# Autodesk Inventor assembly: GP3-100
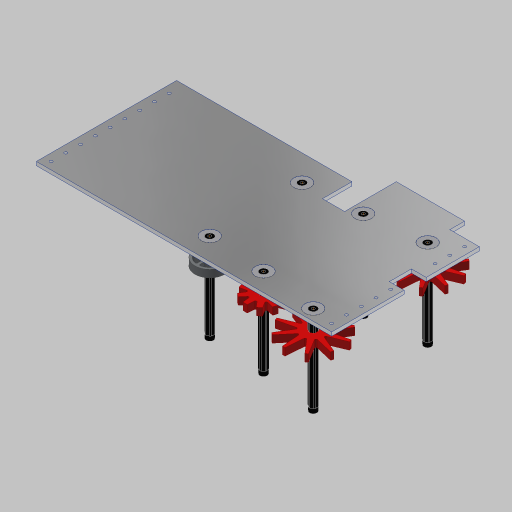
[picture p0: Inventor's stored thumbnail of the model, 512x512]
Saved by Autodesk Inventor 2023.5 (Build 275446000, 446)
## iProperties
Created: 2025-02-22
Part Number: GP3-100
Document SubType Name: Assembly
Designer: slick
Author: slick
## Documents named in this file (7)
- C:\Users\slick\OneDrive\Desktop\2025-ReefScape---CAD\ground intake\GP3\GP3-100.iam
- C:\Users\slick\OneDrive\Desktop\2025-ReefScape---CAD\ground intake\GP3\GP3-001.ipt
- C:\Users\slick\OneDrive\Desktop\2025-ReefScape---CAD\COMMON PARTS\BEARINGS\0_500_ID_x_1_125_OD_x_0_313_WD_Flanged_Bearing_217-2731.ipt
- C:\Users\slick\OneDrive\Desktop\2025-ReefScape---CAD\ground intake\GP3\GP3-002.ipt
- C:\Users\slick\OneDrive\Desktop\2025-ReefScape---CAD\COMMON PARTS\WHEELS\am-0619a .425 Hex Entrapption Star Cut to 4In.ipt
- C:\Users\slick\OneDrive\Desktop\2025-ReefScape---CAD\COMMON PARTS\WHEELS\am-0619a .425 Hex Entrapption Star Cut to 2 half In.ipt
- C:\Users\slick\OneDrive\Desktop\2025-ReefScape---CAD\COMMON PARTS\WHEELS\2_OD_Straight_Flex_Wheel_217-6354.ipt
## Components (19 placed, 6 different names)
1. GP3-001:1 — Insert:1, Insert:2, Insert:3, Mate:6, Insert:4, Insert:5, Insert:6
2. 0_500_ID_x_1_125_OD_x_0_313_WD_Flanged_Bearing_217-2731:1 — Insert:2, Mate:2, Flush:2
3. 0_500_ID_x_1_125_OD_x_0_313_WD_Flanged_Bearing_217-2731:2 — Insert:1, Mate:3, Flush:1
4. 0_500_ID_x_1_125_OD_x_0_313_WD_Flanged_Bearing_217-2731:3 — Insert:3, Mate:1, Flush:3
5. GP3-002:1 — Mate:3, Flush:1, Mate:5
6. GP3-002:2 — Mate:1, Flush:3, Mate:4
7. GP3-002:3 — Mate:2, Flush:2, Mate:8
8. am-0619a .425 Hex Entrapption Star Cut to 4In:2 — Mate:5, Flush:4
9. am-0619a .425 Hex Entrapption Star Cut to 4In:1 — Mate:4, Flush:4, Mate:6, Flush:7
10. 0_500_ID_x_1_125_OD_x_0_313_WD_Flanged_Bearing_217-2731:4 — Insert:4
11. GP3-002:4 — Mate:9
12. am-0619a .425 Hex Entrapption Star Cut to 2 half In:1 — Mate:8, Flush:6
13. am-0619a .425 Hex Entrapption Star Cut to 2 half In:2 — Mate:9, Flush:6, Flush:7, Flush:11
14. 0_500_ID_x_1_125_OD_x_0_313_WD_Flanged_Bearing_217-2731:5 — Insert:5
15. GP3-002:5 — Mate:12
16. 0_500_ID_x_1_125_OD_x_0_313_WD_Flanged_Bearing_217-2731:6 — Insert:6
17. GP3-002:6 — Mate:13
18. 2_OD_Straight_Flex_Wheel_217-6354:1 — Mate:13, Flush:10
19. 2_OD_Straight_Flex_Wheel_217-6354:2 — Mate:12, Flush:10, Flush:11
## Relationships (30: Mate 13, Flush 11, Insert 6)
- Insert:1: GP3-001:1 ↔ 0_500_ID_x_1_125_OD_x_0_313_WD_Flanged_Bearing_217-2731:2
- Insert:2: GP3-001:1 ↔ 0_500_ID_x_1_125_OD_x_0_313_WD_Flanged_Bearing_217-2731:1
- Insert:3: GP3-001:1 ↔ 0_500_ID_x_1_125_OD_x_0_313_WD_Flanged_Bearing_217-2731:3
- Mate:1: 0_500_ID_x_1_125_OD_x_0_313_WD_Flanged_Bearing_217-2731:3 ↔ GP3-002:2
- Mate:2: 0_500_ID_x_1_125_OD_x_0_313_WD_Flanged_Bearing_217-2731:1 ↔ GP3-002:3
- Mate:3: 0_500_ID_x_1_125_OD_x_0_313_WD_Flanged_Bearing_217-2731:2 ↔ GP3-002:1
- Flush:1: 0_500_ID_x_1_125_OD_x_0_313_WD_Flanged_Bearing_217-2731:2 ↔ GP3-002:1
- Flush:2: 0_500_ID_x_1_125_OD_x_0_313_WD_Flanged_Bearing_217-2731:1 ↔ GP3-002:3
- Flush:3: 0_500_ID_x_1_125_OD_x_0_313_WD_Flanged_Bearing_217-2731:3 ↔ GP3-002:2
- Mate:4: GP3-002:2 ↔ am-0619a .425 Hex Entrapption Star Cut to 4In:1
- Mate:5: GP3-002:1 ↔ am-0619a .425 Hex Entrapption Star Cut to 4In:2
- Flush:4: am-0619a .425 Hex Entrapption Star Cut to 4In:2 ↔ am-0619a .425 Hex Entrapption Star Cut to 4In:1
- Mate:6 (25.4 mm): GP3-001:1 ↔ am-0619a .425 Hex Entrapption Star Cut to 4In:1
- [Mate]: 0_500_ID_x_1_125_OD_x_0_313_WD_Flanged_Bearing_217-2731:4 ↔ GP3-002:4
- [Flush]: 0_500_ID_x_1_125_OD_x_0_313_WD_Flanged_Bearing_217-2731:4 ↔ GP3-002:4
- Insert:4: GP3-001:1 ↔ 0_500_ID_x_1_125_OD_x_0_313_WD_Flanged_Bearing_217-2731:4
- Mate:8: GP3-002:3 ↔ am-0619a .425 Hex Entrapption Star Cut to 2 half In:1
- Mate:9: GP3-002:4 ↔ am-0619a .425 Hex Entrapption Star Cut to 2 half In:2
- Flush:6: am-0619a .425 Hex Entrapption Star Cut to 2 half In:1 ↔ am-0619a .425 Hex Entrapption Star Cut to 2 half In:2
- Flush:7: am-0619a .425 Hex Entrapption Star Cut to 4In:1 ↔ am-0619a .425 Hex Entrapption Star Cut to 2 half In:2
- [Mate]: 0_500_ID_x_1_125_OD_x_0_313_WD_Flanged_Bearing_217-2731:5 ↔ GP3-002:5
- [Flush]: 0_500_ID_x_1_125_OD_x_0_313_WD_Flanged_Bearing_217-2731:5 ↔ GP3-002:5
- [Mate]: 0_500_ID_x_1_125_OD_x_0_313_WD_Flanged_Bearing_217-2731:6 ↔ GP3-002:6
- [Flush]: 0_500_ID_x_1_125_OD_x_0_313_WD_Flanged_Bearing_217-2731:6 ↔ GP3-002:6
- Insert:5: GP3-001:1 ↔ 0_500_ID_x_1_125_OD_x_0_313_WD_Flanged_Bearing_217-2731:5
- Insert:6: GP3-001:1 ↔ 0_500_ID_x_1_125_OD_x_0_313_WD_Flanged_Bearing_217-2731:6
- Mate:12: GP3-002:5 ↔ 2_OD_Straight_Flex_Wheel_217-6354:2
- Mate:13: GP3-002:6 ↔ 2_OD_Straight_Flex_Wheel_217-6354:1
- Flush:10: 2_OD_Straight_Flex_Wheel_217-6354:1 ↔ 2_OD_Straight_Flex_Wheel_217-6354:2
- Flush:11: am-0619a .425 Hex Entrapption Star Cut to 2 half In:2 ↔ 2_OD_Straight_Flex_Wheel_217-6354:2
## Named parameters: d26_d10 = 0 mm, d27_d7 = 0 mm, d33_d26_d10 = 0 mm, d34_d27_d7 = 0 mm, d35_d33_d26_d10 = 0 mm, d36_d34_d27_d7 = 0 mm
